# Autodesk Inventor assembly: ChassisMainTeil
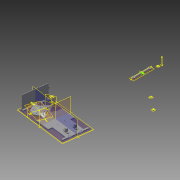
[picture p0: Inventor's stored thumbnail of the model, 180x180]
Saved by Autodesk Inventor 2015 (Build 190159000, 159)
## iProperties
Created: 2018-11-02
Part Number: ChassisMainTeil
Document SubType Name: Assembly
Designer: Boris
Author: Boris
## Documents named in this file (8)
- D:\Wisag Hiserv\HiSERV Smart Drive\WorkOrder\3D - Teile\ChassisMainTeil.iam
- D:\Wisag Hiserv\HiSERV Smart Drive\WorkOrder\3D - Teile\Chassis.ipt
- D:\Wisag Hiserv\HiSERV Smart Drive\WorkOrder\3D - Teile\ChassisOberTeil.ipt
- D:\Wisag Hiserv\HiSERV Smart Drive\WorkOrder\3D - Teile\LenkStange.ipt
- D:\Wisag Hiserv\HiSERV Smart Drive\WorkOrder\3D - Teile\LenkStangeSicherung.ipt
- D:\Wisag Hiserv\HiSERV Smart Drive\WorkOrder\3D - Teile\LenkungStütze.ipt
- D:\Wisag Hiserv\HiSERV Smart Drive\WorkOrder\3D - Teile\LenkungTeil1.ipt
- D:\Wisag Hiserv\HiSERV Smart Drive\WorkOrder\3D - Teile\KugelLager.ipt
## Components (13 placed, 7 different names)
1. Chassis:1 — Einfügen:1, Einfügen:2, Drehbar:1
2. ChassisOberTeil:1 — Einfügen:3, Drehbar:3
3. LenkStange:1
4. LenkStangeSicherung:1
5. LenkungStütze:1
6. LenkungTeil1:1 — Drehbar:1, Drehbar:3
7. KugelLager:1 — Einfügen:3
8. KugelLager:2
9. KugelLager:3 — Einfügen:1
10. KugelLager:4
11. KugelLager:5 — Einfügen:2, Drehbar:2
12. KugelLager:6 — Drehbar:4
13. LenkungTeil1:2 — Drehbar:2, Drehbar:4
## Relationships (7: RevoluteJoint 4, Insert 3)
- Einfügen:1 [Insert] (-4 mm): Chassis:1 ↔ KugelLager:3
- Einfügen:2 [Insert]: Chassis:1 ↔ KugelLager:5
- Drehbar:1 [RevoluteJoint]: Chassis:1 ↔ LenkungTeil1:1
- Drehbar:2 [RevoluteJoint]: KugelLager:5 ↔ LenkungTeil1:2
- Einfügen:3 [Insert] (3 mm): ChassisOberTeil:1 ↔ KugelLager:1
- Drehbar:3 [RevoluteJoint]: ChassisOberTeil:1 ↔ LenkungTeil1:1
- Drehbar:4 [RevoluteJoint]: KugelLager:6 ↔ LenkungTeil1:2
